# Autodesk Inventor assembly: Table
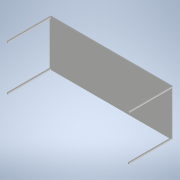
[picture p0: Inventor's stored thumbnail of the model, 180x180]
Saved by Autodesk Inventor 2020 (Build 240168000, 168)
## iProperties
Created: 2019-11-09
Part Number: Table
Document SubType Name: Assembly
Designer: nicoc
Author: nicoc
## Documents named in this file (3)
- D:\03_Bachelor\Semester_5\pro5E\Stand\CAD\Version2\Table\Table.iam
- D:\03_Bachelor\Semester_5\pro5E\Stand\CAD\Version2\Table\Tabletop.ipt
- D:\03_Bachelor\Semester_5\pro5E\Stand\CAD\Version2\Table\TableLeg.ipt
## Components (5 placed, 2 different names)
1. Tabletop:1 — Mate:1, Flush:1, Flush:2, Flush:3, Flush:4, Mate:2, Mate:3, Flush:5, Flush:6, Mate:4, Flush:7, Flush:8
2. TableLeg:1 — Mate:1, Flush:1, Flush:2
3. TableLeg:2 — Flush:3, Flush:4, Mate:2
4. TableLeg:3 — Mate:3, Flush:5, Flush:6
5. TableLeg:4 — Mate:4, Flush:7, Flush:8
## Relationships (12: Flush 8, Mate 4)
- Mate:1: Tabletop:1 ↔ TableLeg:1
- Flush:1: Tabletop:1 ↔ TableLeg:1
- Flush:2: Tabletop:1 ↔ TableLeg:1
- Flush:3: Tabletop:1 ↔ TableLeg:2
- Flush:4: Tabletop:1 ↔ TableLeg:2
- Mate:2: Tabletop:1 ↔ TableLeg:2
- Mate:3: Tabletop:1 ↔ TableLeg:3
- Flush:5: Tabletop:1 ↔ TableLeg:3
- Flush:6: Tabletop:1 ↔ TableLeg:3
- Mate:4: Tabletop:1 ↔ TableLeg:4
- Flush:7: Tabletop:1 ↔ TableLeg:4
- Flush:8: Tabletop:1 ↔ TableLeg:4
